# Autodesk Inventor assembly: Assembly1
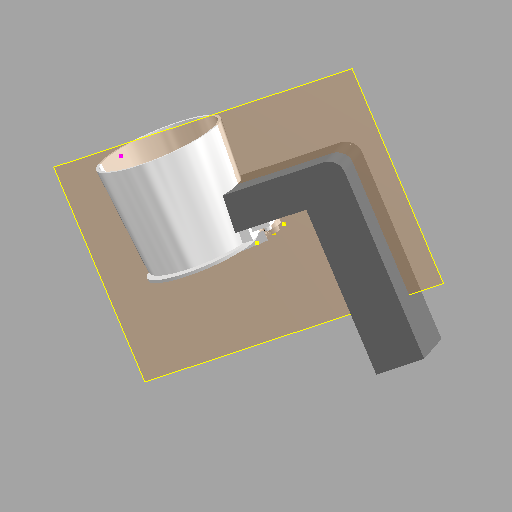
[picture p0: Inventor's stored thumbnail of the model, 512x512]
Saved by Autodesk Inventor 2025.3 (Build 293356000, 356)
## iProperties
Created: 2026-03-06
Part Number: Assembly1
Document SubType Name: Assembly
Designer: Youssef Makhlouf
Author: Youssef Makhlouf
## Documents named in this file (5)
- C:\Ayman\Inventor Projects\Lifting Mechanism\Assembly1.iam
- C:\Ayman\Inventor Projects\Lifting Mechanism\Part1'.ipt
- C:\Ayman\Inventor Projects\Lifting Mechanism\Part2.ipt
- C:\Ayman\Inventor Projects\Lifting Mechanism\Part3.ipt
- C:\Ayman\Inventor Projects\Lifting Mechanism\Cover.ipt
## Components (4 placed, 4 different names)
1. Part3:1 — Mate:11, Mate:13, Mate:14, Flush:1
2. Part1':1 — Mate:6, Mate:7, Mate:11, Mate:13, Mate:14
3. Part2:1 — Mate:6, Mate:7, Mate:15, Mate:16, Mate:17
4. Cover:1 — Mate:15, Mate:16, Mate:17
## Relationships (9: Mate 8, Flush 1)
- Mate:6: Part1':1 ↔ Part2:1
- Mate:7: Part1':1 ↔ Part2:1
- Mate:11: Part3:1 ↔ Part1':1
- Mate:13: Part3:1 ↔ Part1':1
- Mate:14 (1 mm): Part3:1 ↔ Part1':1
- Mate:15 (1 mm): Part2:1 ↔ Cover:1
- Mate:16 (1 mm): Part2:1 ↔ Cover:1
- Mate:17 (1 mm): Part2:1 ↔ Cover:1
- Flush:1 (-18.4531 mm): Part3:1
## Named parameters: Finish1_Area = 235.675, Finish1_Thickness = 0.05 mm, Finish2_Area = 273.978, Finish2_Thickness = 0.05 mm
note: some values were not read from the file. Shown as the stored number, unit unknown: "Finish1_Area", "Finish2_Area".
